# Autodesk Inventor assembly: HbthumbU01
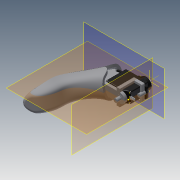
[picture p0: Inventor's stored thumbnail of the model, 180x180]
Saved by Autodesk Inventor 2015 SP1 (Build 190203100, 203)
## iProperties
Created: 2015-02-19
Part Number: HbthumbU01
Document SubType Name: Assembly
Designer: Yamaura
Author: Yamaura
## Documents named in this file (4)
- C:\Users\Yamaura\Google ドライブ\exiii\3D\150405HackBerry\00_Latest\HbthumbU01.iam
- C:\Users\Yamaura\Google ドライブ\exiii\3D\150405HackBerry\00_Latest\ASV-15MG.ipt
- C:\Users\Yamaura\Google ドライブ\exiii\3D\150405HackBerry\00_Latest\ScrewM2L8.ipt
- C:\Users\Yamaura\Google ドライブ\exiii\3D\150405HackBerry\00_Latest\Hbthumb03.ipt
## Components (4 placed, 3 different names)
1. ASV-15MG:1 — フラッシュ:1, メイト:1, 角度:1, メイト:4, メイト:5, メイト:6, メイト:7
2. ScrewM2L8:1 — メイト:4, メイト:5
3. ScrewM2L8:2 — メイト:6, メイト:7
4. Hbthumb03:1
## Relationships (7: Mate 5, Flush 1, Angle 1)
- フラッシュ:1 [Flush]: ASV-15MG:1
- メイト:1 [Mate]: ASV-15MG:1
- 角度:1 [Angle] (0 deg): ASV-15MG:1
- メイト:4 [Mate]: ASV-15MG:1 ↔ ScrewM2L8:1
- メイト:5 [Mate]: ASV-15MG:1 ↔ ScrewM2L8:1
- メイト:6 [Mate]: ASV-15MG:1 ↔ ScrewM2L8:2
- メイト:7 [Mate]: ASV-15MG:1 ↔ ScrewM2L8:2
